# Autodesk Inventor assembly: ASY leg1
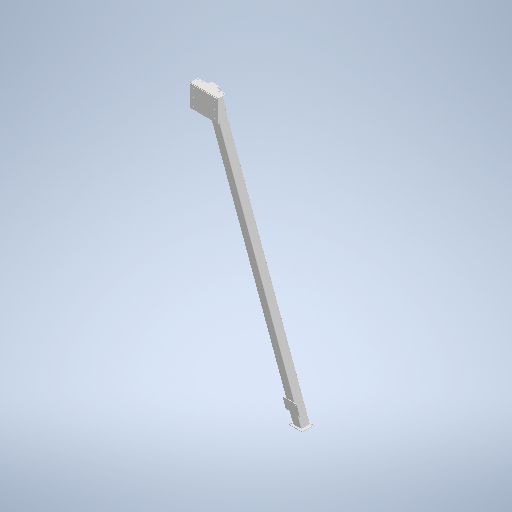
[picture p0: Inventor's stored thumbnail of the model, 512x512]
Saved by Autodesk Inventor 2025 (Build 290162010, 162A)
## iProperties
Created: 2024-07-08
Part Number: ASY leg1
Document SubType Name: Assembly
Designer: admin
Author: admin
## Documents named in this file (6)
- C:\Users\user\YandexDisk\домашниий пк\Inventor\Workshop\оборудование\Goat 2\leg 1\ASY leg1.iam
- C:\Users\user\YandexDisk\домашниий пк\Inventor\Workshop\оборудование\Goat 2\Сrane plate 3.ipt
- C:\Users\user\YandexDisk\домашниий пк\Inventor\Workshop\оборудование\Goat 2\Сrane plate 2.ipt
- C:\Users\user\YandexDisk\домашниий пк\Inventor\Workshop\оборудование\Goat 2\Сrane plate 4.ipt
- C:\Users\user\YandexDisk\домашниий пк\Inventor\Workshop\оборудование\Goat 2\Stand.ipt
- C:\Users\user\YandexDisk\домашниий пк\Inventor\Workshop\оборудование\Goat 2\Сrane plate 6.ipt
## Components (7 placed, 6 different names)
1. Сrane plate 3.ipt:2
2. Сrane plate 2.ipt:2
3. Сrane plate 4.ipt:3
4. Сrane plate 4.ipt:4
5. Stand.ipt:2
6. Сrane plate 6.ipt:2
7. Сrane plate 6:3
## Relationships (11: Mate 8, WeldJoint 2, Flush 1)
- [WeldJoint]: Сrane plate 3.ipt:2 ↔ Сrane plate 2.ipt:2
- [Mate]: Сrane plate 3.ipt:2 ↔ Сrane plate 4.ipt:3
- [Mate]: Сrane plate 2.ipt:2 ↔ Сrane plate 4.ipt:3
- [Mate]: Сrane plate 3.ipt:2 ↔ Сrane plate 4.ipt:4
- [Mate]: Сrane plate 2.ipt:2 ↔ Сrane plate 4.ipt:4
- [Mate]: Сrane plate 2.ipt:2 ↔ Stand.ipt:2
- [Mate]: Сrane plate 4.ipt:4 ↔ Stand.ipt:2
- [Flush]: Сrane plate 4.ipt:3 ↔ Stand.ipt:2
- [Mate]: Stand.ipt:2 ↔ Сrane plate 6.ipt:2
- [Mate] (-200 mm): Stand.ipt:2 ↔ Сrane plate 6.ipt:2
- [WeldJoint]: Stand.ipt:2 ↔ Сrane plate 6:3
